# Autodesk Inventor assembly: MECANISMO DE COMPACTADO V2
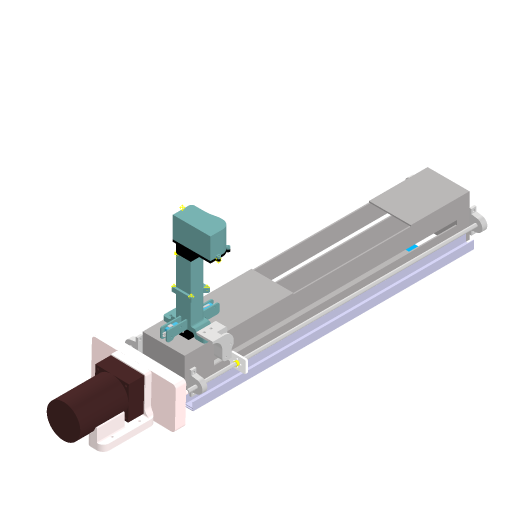
[picture p0: Inventor's stored thumbnail of the model, 512x512]
Saved by Autodesk Inventor 2024 (Build 280153000, 153)
## iProperties
Created: 2024-08-15
Part Number: MECANISMO DE COMPACTADO V2
Document SubType Name: Assembly
Designer: Jhuliams
Author: Jhuliams
## Documents named in this file (14)
- C:\Users\Jhuliams\Documents\GitHub\RECICLADOR_MODELO_3D\MECANISMO DE COMPACTADO\MECANISMO DE COMPACTADO V2.iam
- C:\Users\Jhuliams\Documents\GitHub\RECICLADOR_MODELO_3D\MECANISMO DE COMPACTADO\GUIA_CUADRADA.ipt
- C:\Users\Jhuliams\Documents\GitHub\RECICLADOR_MODELO_3D\MECANISMO DE COMPACTADO\TUERCA DE HUSILLO.ipt
- C:\Users\Jhuliams\Documents\GitHub\RECICLADOR_MODELO_3D\MECANISMO DE COMPACTADO\TORNILLO DEPOTENCIA.ipt
- C:\Users\Jhuliams\Documents\GitHub\RECICLADOR_MODELO_3D\MECANISMO DE COMPACTADO\RODAMIENTO DE TORNILLO.ipt
- C:\Users\Jhuliams\Documents\GitHub\RECICLADOR_MODELO_3D\MECANISMO DE COMPACTADO\SOPORTE DEL MOTOR.ipt
- C:\Users\Jhuliams\Documents\GitHub\RECICLADOR_MODELO_3D\MECANISMO DE COMPACTADO\MOTOR DC.ipt
- C:\Users\Jhuliams\Documents\GitHub\RECICLADOR_MODELO_3D\MECANISMO DE COMPACTADO\CAJA REDUCTORA.ipt
- C:\Users\Jhuliams\Documents\GitHub\RECICLADOR_MODELO_3D\MECANISMO DE COMPACTADO\GUIA_CANALETA.ipt
- C:\Users\Jhuliams\Documents\GitHub\RECICLADOR_MODELO_3D\MECANISMO DE COMPACTADO\CANALETA_PLANA.ipt
- C:\Users\Jhuliams\Documents\GitHub\RECICLADOR_MODELO_3D\ACTUADOR_PARA_EMPUJAR_HACIA_ABAJO\ACTUADOR_LINEAL.iam
- C:\Users\Jhuliams\Documents\GitHub\RECICLADOR_MODELO_3D\MECANISMO DE COMPACTADO\TAPA QUE DESPLAZA CON TORNILLOS.ipt
- C:\Users\Jhuliams\Documents\GitHub\RECICLADOR_MODELO_3D\MECANISMO DE COMPACTADO\SOPORTE_FDC.ipt
- C:\Users\Jhuliams\Documents\GitHub\RECICLADOR_MODELO_3D\ACTUADOR_PARA_EMPUJAR_HACIA_ABAJO\FIN_DE_CARRERA.ipt
## Components (21 placed, 13 different names)
1. GUIA_CUADRADA:1 — Flush:2, Mate:12, Flush:4, Flush:5, Flush:7, Flush:8, Mate:24, Flush:9, Mate:27, Flush:11, Flush:12, Mate:32, Mate:33, Mate:34, Mate:36
2. TUERCA DE HUSILLO:1 — Mate:3, Mate:35, Mate:37
3. TUERCA DE HUSILLO:2 — Mate:4, Mate:38
4. TORNILLO DEPOTENCIA:1 — Mate:3, Flush:1, Mate:11, Mate:14, Flush:7, Mate:22, Mate:23
5. TORNILLO DEPOTENCIA:2 — Mate:4, Flush:1, Mate:13, Mate:15, Mate:21
6. RODAMIENTO DE TORNILLO:1 — Mate:11, Flush:2, Mate:12, Flush:3
7. RODAMIENTO DE TORNILLO:2 — Mate:14, Flush:4
8. RODAMIENTO DE TORNILLO:3 — Mate:15, Flush:5
9. RODAMIENTO DE TORNILLO:4 — Mate:13, Flush:3
10. SOPORTE DEL MOTOR:1 — Mate:16, Mate:17, Mate:18, Mate:20, Flush:6
11. MOTOR DC:1 — Mate:16, Mate:17, Mate:18, Mate:19
12. CAJA REDUCTORA:1 — Mate:19, Mate:20, Flush:6, Mate:21, Mate:22, Mate:23
13. GUIA_CANALETA:1 — Flush:8, Mate:24, Flush:9, Mate:25, Flush:10, Mate:26
14. GUIA_CANALETA:2 — Mate:25, Flush:10, Mate:26
15. GUIA_CANALETA:3 — Mate:27, Flush:11, Flush:12, Flush:13, Mate:28, Mate:29
16. GUIA_CANALETA:4 — Flush:13, Mate:28, Mate:29, Mate:30, Mate:31
17. CANALETA_PLANA:1 — Mate:30, Mate:31
18. ACTUADOR_LINEAL:1 [sub-assembly] — Mate:32, Mate:33, Mate:34, Mate:39, Mate:40, Mate:41
19. TAPA QUE DESPLAZA CON TORNILLOS:1 — Mate:35, Mate:36, Mate:37, Mate:38
20. SOPORTE_FDC:1 — Mate:39, Mate:40, Mate:41, Mate:42, Mate:43, Mate:44
21. FIN_DE_CARRERA:1 — Mate:42, Mate:43, Mate:44
## Relationships (49: Mate 36, Flush 13)
- Mate:3: TUERCA DE HUSILLO:1 ↔ TORNILLO DEPOTENCIA:1
- Mate:4: TUERCA DE HUSILLO:2 ↔ TORNILLO DEPOTENCIA:2
- Flush:1: TORNILLO DEPOTENCIA:1 ↔ TORNILLO DEPOTENCIA:2
- Mate:11: TORNILLO DEPOTENCIA:1 ↔ RODAMIENTO DE TORNILLO:1
- Flush:2: GUIA_CUADRADA:1 ↔ RODAMIENTO DE TORNILLO:1
- Mate:12 (11.5 mm): GUIA_CUADRADA:1 ↔ RODAMIENTO DE TORNILLO:1
- Mate:13: TORNILLO DEPOTENCIA:2 ↔ RODAMIENTO DE TORNILLO:4
- Mate:14: TORNILLO DEPOTENCIA:1 ↔ RODAMIENTO DE TORNILLO:2
- Mate:15: TORNILLO DEPOTENCIA:2 ↔ RODAMIENTO DE TORNILLO:3
- Flush:3: RODAMIENTO DE TORNILLO:1 ↔ RODAMIENTO DE TORNILLO:4
- Flush:4: GUIA_CUADRADA:1 ↔ RODAMIENTO DE TORNILLO:2
- Flush:5: GUIA_CUADRADA:1 ↔ RODAMIENTO DE TORNILLO:3
- Mate:16: SOPORTE DEL MOTOR:1 ↔ MOTOR DC:1
- Mate:17: SOPORTE DEL MOTOR:1 ↔ MOTOR DC:1
- Mate:18: SOPORTE DEL MOTOR:1 ↔ MOTOR DC:1
- Mate:19: MOTOR DC:1 ↔ CAJA REDUCTORA:1
- Mate:20: SOPORTE DEL MOTOR:1 ↔ CAJA REDUCTORA:1
- Flush:6: SOPORTE DEL MOTOR:1 ↔ CAJA REDUCTORA:1
- Flush:7: GUIA_CUADRADA:1 ↔ TORNILLO DEPOTENCIA:1
- Mate:21: TORNILLO DEPOTENCIA:2 ↔ CAJA REDUCTORA:1
- Mate:22: TORNILLO DEPOTENCIA:1 ↔ CAJA REDUCTORA:1
- Mate:23 (2 mm): TORNILLO DEPOTENCIA:1 ↔ CAJA REDUCTORA:1
- Flush:8: GUIA_CUADRADA:1 ↔ GUIA_CANALETA:1
- Mate:24: GUIA_CUADRADA:1 ↔ GUIA_CANALETA:1
- Flush:9: GUIA_CUADRADA:1 ↔ GUIA_CANALETA:1
- Mate:25: GUIA_CANALETA:1 ↔ GUIA_CANALETA:2
- Flush:10: GUIA_CANALETA:1 ↔ GUIA_CANALETA:2
- Mate:26 (3 mm): GUIA_CANALETA:1 ↔ GUIA_CANALETA:2
- Mate:27: GUIA_CUADRADA:1 ↔ GUIA_CANALETA:3
- Flush:11: GUIA_CUADRADA:1 ↔ GUIA_CANALETA:3
- Flush:12: GUIA_CUADRADA:1 ↔ GUIA_CANALETA:3
- Flush:13: GUIA_CANALETA:3 ↔ GUIA_CANALETA:4
- Mate:28: GUIA_CANALETA:3 ↔ GUIA_CANALETA:4
- Mate:29 (3 mm): GUIA_CANALETA:3 ↔ GUIA_CANALETA:4
- Mate:30: GUIA_CANALETA:4 ↔ CANALETA_PLANA:1
- Mate:31 (4 mm): GUIA_CANALETA:4 ↔ CANALETA_PLANA:1
- Mate:32: GUIA_CUADRADA:1 ↔ ACTUADOR_LINEAL:1
- Mate:33: GUIA_CUADRADA:1 ↔ ACTUADOR_LINEAL:1
- Mate:34: GUIA_CUADRADA:1 ↔ ACTUADOR_LINEAL:1
- Mate:35: TUERCA DE HUSILLO:1 ↔ TAPA QUE DESPLAZA CON TORNILLOS:1
- Mate:36 (0.5 mm): GUIA_CUADRADA:1 ↔ TAPA QUE DESPLAZA CON TORNILLOS:1
- Mate:37: TUERCA DE HUSILLO:1 ↔ TAPA QUE DESPLAZA CON TORNILLOS:1
- Mate:38: TUERCA DE HUSILLO:2 ↔ TAPA QUE DESPLAZA CON TORNILLOS:1
- Mate:39: ACTUADOR_LINEAL:1 ↔ SOPORTE_FDC:1
- Mate:40: ACTUADOR_LINEAL:1 ↔ SOPORTE_FDC:1
- Mate:41: ACTUADOR_LINEAL:1 ↔ SOPORTE_FDC:1
- Mate:42: SOPORTE_FDC:1 ↔ FIN_DE_CARRERA:1
- Mate:43: SOPORTE_FDC:1 ↔ FIN_DE_CARRERA:1
- Mate:44 (0.5 mm): SOPORTE_FDC:1 ↔ FIN_DE_CARRERA:1
